# Autodesk Inventor assembly: Hinge Assembly
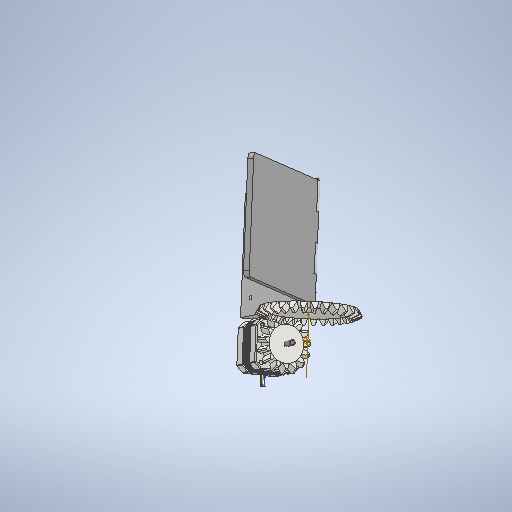
[picture p0: Inventor's stored thumbnail of the model, 512x512]
Saved by Autodesk Inventor 2025.1 (Build 291241000, 241)
## iProperties
Created: 2024-10-22
Part Number: Hinge Assembly
Document SubType Name: Assembly
Designer: vedan
Author: vedan
## Documents named in this file (5)
- C:\Users\vedan\OneDrive\Desktop\Engineer 1P13\Design Studio\Project 1\files\Hinge Assembly.iam
- C:\Users\vedan\OneDrive\Desktop\Engineer 1P13\Design Studio\Project 1\files\Rod.ipt
- C:\Users\vedan\OneDrive\Desktop\Engineer 1P13\Design Studio\Project 1\files\Hinge2.ipt
- C:\Users\vedan\OneDrive\Desktop\Engineer 1P13\Design Studio\Project 1\files\bevel gear system.iam
- C:\Users\vedan\OneDrive\Desktop\Engineer 1P13\Design Studio\Project 1\files\Hinge.ipt
## Components (4 placed, 4 different names)
1. Rod:2 — Mate:3, Mate:8, Mate:10, Angle:1, Angle:4, Flush:1, Mate:18, Angle:6
2. Hinge2:1 — Mate:3, Mate:10, Mate:15, Angle:4, Angle:5, Mate:16, Mate:17
3. bevel gear system:1 [sub-assembly] — Mate:8, Angle:1, Flush:1, Angle:5
4. Hinge:4 — Mate:15, Mate:16, Mate:17, Mate:18, Angle:6
## Relationships (12: Mate 7, Angle 4, Flush 1)
- Mate:3: Rod:2 ↔ Hinge2:1
- Mate:8: Rod:2 ↔ bevel gear system:1
- Mate:10: Rod:2 ↔ Hinge2:1
- Angle:1 (180 deg): Rod:2 ↔ bevel gear system:1
- Mate:15: Hinge2:1 ↔ Hinge:4
- Angle:4 (0 deg): Rod:2 ↔ Hinge2:1
- Flush:1: Rod:2 ↔ bevel gear system:1
- Angle:5 (0 deg): Hinge2:1 ↔ bevel gear system:1
- Mate:16: Hinge2:1 ↔ Hinge:4
- Mate:17: Hinge2:1 ↔ Hinge:4
- Mate:18: Rod:2 ↔ Hinge:4
- Angle:6 (0 deg): Rod:2 ↔ Hinge:4
